# Autodesk Inventor assembly: Ontvanger
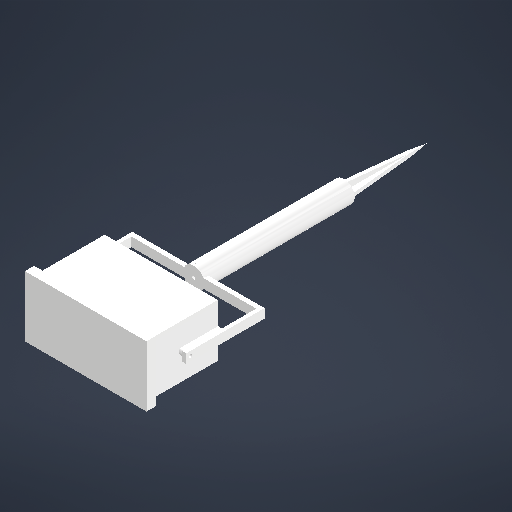
[picture p0: Inventor's stored thumbnail of the model, 512x512]
Saved by Autodesk Inventor 2026.2 (Build 302298000, 298)
## iProperties
Created: 2026-05-05
Part Number: Ontvanger
Document SubType Name: Assembly
Designer: Gameb
Author: Gameb
## Documents named in this file (6)
- C:\Users\Gameb\OneDrive - Stichting Hogeschool Utrecht\Jaar 3\Periode C&D\Quest\11- secor ontwikkeling\3D ontwerp\Ontvanger.iam
- C:\Users\Gameb\OneDrive - Stichting Hogeschool Utrecht\Jaar 3\Periode C&D\Quest\11- secor ontwikkeling\3D ontwerp\Tussen stuk V1.1.ipt
- C:\Users\Gameb\OneDrive - Stichting Hogeschool Utrecht\Jaar 3\Periode C&D\Quest\11- secor ontwikkeling\3D ontwerp\Prikker V1.1.ipt
- C:\Users\Gameb\OneDrive - Stichting Hogeschool Utrecht\Jaar 3\Periode C&D\Quest\11- secor ontwikkeling\3D ontwerp\Bakje sensor.ipt
- C:\Users\Gameb\OneDrive - Stichting Hogeschool Utrecht\Jaar 3\Periode C&D\Quest\11- secor ontwikkeling\3D ontwerp\Deksel sensor.ipt
- C:\Users\Gameb\OneDrive - Stichting Hogeschool Utrecht\Jaar 3\Periode C&D\Quest\11- secor ontwikkeling\3D ontwerp\Sensor houder.ipt
## Components (5 placed, 5 different names)
1. Prikker V1.1:1 — Mate:4
2. Bakje sensor:1 — Mate:1, Mate:2
3. Deksel sensor:1 — Mate:1
4. Sensor houder:1 — Mate:2, Mate:3
5. Tussen stuk V1.1:1 — Mate:3, Mate:4
## Relationships (4: Mate 4)
- Mate:1: Bakje sensor:1 ↔ Deksel sensor:1
- Mate:2: Bakje sensor:1 ↔ Sensor houder:1
- Mate:3: Sensor houder:1 ↔ Tussen stuk V1.1:1
- Mate:4: Prikker V1.1:1 ↔ Tussen stuk V1.1:1
